# Autodesk Inventor assembly: Adquisicion señales
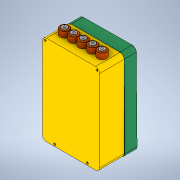
[picture p0: Inventor's stored thumbnail of the model, 180x180]
Saved by Autodesk Inventor 2020 (Build 240168000, 168)
## iProperties
Created: 2022-05-21
Part Number: Adquisicion señales
Document SubType Name: Assembly
Designer: juanc
Author: juanc
## Documents named in this file (7)
- C:\Users\juanc\Desktop\ProyectoIntegrador\3D Model\Adquisicion señales.iam
- C:\Users\juanc\Desktop\ProyectoIntegrador\3D Model\carcasa inferior.ipt
- C:\Users\juanc\Desktop\ProyectoIntegrador\3D Model\pilas y portapilas.iam
- C:\Users\juanc\Desktop\ProyectoIntegrador\3D Model\arduino nano.iam
- C:\Users\juanc\Desktop\ProyectoIntegrador\3D Model\pcb 3d\PCB Final un canal.iam
- C:\Users\juanc\Desktop\ProyectoIntegrador\3D Model\Banana Hembra.ipt
- C:\Users\juanc\Desktop\ProyectoIntegrador\3D Model\CARCASA SUPERIOR.ipt
## Components (11 placed, 6 different names)
1. carcasa inferior:1 — Rotational:1, Mate:1, Mate:2, Rotational:3, Rotational:2, Rotational:4, Rotational:5, Rotational:6, Rotational:7
2. pilas y portapilas:1 [sub-assembly] — Rotational:1
3. arduino nano:1 [sub-assembly]
4. PCB Final un canal:1 [sub-assembly] — Mate:2
5. PCB Final un canal:2 [sub-assembly] — Mate:1
6. Banana Hembra:1 — Rotational:3
7. Banana Hembra:2 — Rotational:2
8. Banana Hembra:3 — Rotational:4
9. Banana Hembra:5 — Rotational:5
10. Banana Hembra:6 — Rotational:6
11. CARCASA SUPERIOR:1 — Rotational:7
## Relationships (9: RevoluteJoint 7, Mate 2)
- Rotational:1 [RevoluteJoint]: carcasa inferior:1 ↔ pilas y portapilas:1
- Mate:1: carcasa inferior:1 ↔ PCB Final un canal:2
- Mate:2: carcasa inferior:1 ↔ PCB Final un canal:1
- Rotational:3 [RevoluteJoint]: carcasa inferior:1 ↔ Banana Hembra:1
- Rotational:2 [RevoluteJoint]: carcasa inferior:1 ↔ Banana Hembra:2
- Rotational:4 [RevoluteJoint]: carcasa inferior:1 ↔ Banana Hembra:3
- Rotational:5 [RevoluteJoint]: carcasa inferior:1 ↔ Banana Hembra:5
- Rotational:6 [RevoluteJoint]: carcasa inferior:1 ↔ Banana Hembra:6
- Rotational:7 [RevoluteJoint]: carcasa inferior:1 ↔ CARCASA SUPERIOR:1
